# Autodesk Inventor assembly: atx-layout
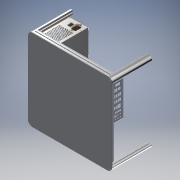
[picture p0: Inventor's stored thumbnail of the model, 180x180]
Saved by Autodesk Inventor 2018 (Build 220112000, 112)
## iProperties
Created: 2021-04-25
Part Number: atx-layout
Document SubType Name: Assembly
Designer: gisen
Author: gisen
## Documents named in this file (9)
- C:\Users\sbbgi\Documents\GitHub\eatx_case\atx\atx-layout.iam
- C:\Users\sbbgi\Documents\GitHub\eatx_case\atx\resources\motherboard\dummy_atx.iam
- C:\Users\sbbgi\Documents\GitHub\eatx_case\atx\parts\right_panel_atx.ipt
- C:\Users\sbbgi\Documents\GitHub\eatx_case\atx\parts\s340.ipt
- 00000010.ipt
- C:\Users\sbbgi\Documents\GitHub\eatx_case\atx\parts\r150.ipt
- 00000008.ipt
- C:\Users\sbbgi\Documents\GitHub\eatx_case\atx\resources\powersupply\ATX Power Supply v1.0.iam
- C:\Users\sbbgi\Documents\GitHub\eatx_case\atx\parts\inner_panel.ipt
## Components (10 placed, 6 different names)
1. dummy_atx:1 [sub-assembly] — Mate:15, Angle:1
2. right_panel_atx:1 — Mate:1, Mate:2, Tangent:1, Mate:3, Mate:4, Tangent:2, Mate:5, Mate:6, Tangent:3, Mate:7, Mate:8, Tangent:4, Mate:10, Flush:1, Mate:12, Flush:2
3. 00000010:1 — Mate:10, Mate:11, Flush:1
4. 00000008:1 — Mate:1, Mate:2, Tangent:1
5. 00000008:2 — Mate:5, Mate:6, Tangent:3
6. 00000008:3 — Mate:7, Mate:8, Tangent:4, Mate:13
7. 00000008:4 — Mate:3, Mate:4, Tangent:2, Mate:11
8. 00000010:2 — Mate:12, Flush:2, Mate:13, Mate:14, Flush:4
9. ATX Power Supply v1.0:1 [sub-assembly] — Flush:5
10. inner_panel:1 — Mate:14, Flush:4, Mate:15, Angle:1, Flush:5
## Relationships (23: Mate 14, Tangent 4, Flush 4, Angle 1)
- Mate:1: right_panel_atx:1 ↔ 00000008:1
- Mate:2: right_panel_atx:1 ↔ 00000008:1
- Tangent:1: right_panel_atx:1 ↔ 00000008:1
- Mate:3: right_panel_atx:1 ↔ 00000008:4
- Mate:4: right_panel_atx:1 ↔ 00000008:4
- Tangent:2: right_panel_atx:1 ↔ 00000008:4
- Mate:5: right_panel_atx:1 ↔ 00000008:2
- Mate:6: right_panel_atx:1 ↔ 00000008:2
- Tangent:3: right_panel_atx:1 ↔ 00000008:2
- Mate:7: right_panel_atx:1 ↔ 00000008:3
- Mate:8: right_panel_atx:1 ↔ 00000008:3
- Tangent:4: right_panel_atx:1 ↔ 00000008:3
- Mate:10: right_panel_atx:1 ↔ 00000010:1
- Mate:11: 00000010:1 ↔ 00000008:4
- Flush:1: right_panel_atx:1 ↔ 00000010:1
- Mate:12: right_panel_atx:1 ↔ 00000010:2
- Flush:2: right_panel_atx:1 ↔ 00000010:2
- Mate:13: 00000008:3 ↔ 00000010:2
- Mate:14: 00000010:2 ↔ inner_panel:1
- Flush:4: 00000010:2 ↔ inner_panel:1
- Mate:15: dummy_atx:1 ↔ inner_panel:1
- Angle:1 (0 deg): dummy_atx:1 ↔ inner_panel:1
- Flush:5: ATX Power Supply v1.0:1 ↔ inner_panel:1
